# Autodesk Inventor assembly: mecanismo
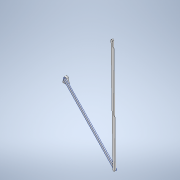
[picture p0: Inventor's stored thumbnail of the model, 180x180]
Saved by Autodesk Inventor 2021 (Build 250183000, 183)
## iProperties
Created: 2021-07-19
Part Number: mecanismo
Document SubType Name: Assembly
Designer: Leonardo Fabio Mercado Benítez
Author: Leonardo Fabio Mercado Benítez
## Documents named in this file (4)
- C:\Users\leo7s\Documents\Universidad\02 Servomecanismos\07 Proyecto Final\proyecto_final_Servomecanismos\02 CADs\mecanismo.iam
- C:\Users\leo7s\Documents\Universidad\02 Servomecanismos\07 Proyecto Final\proyecto_final_Servomecanismos\02 CADs\base.ipt
- C:\Users\leo7s\Documents\Universidad\02 Servomecanismos\07 Proyecto Final\proyecto_final_Servomecanismos\02 CADs\eslabon_1.ipt
- C:\Users\leo7s\Documents\Universidad\02 Servomecanismos\07 Proyecto Final\proyecto_final_Servomecanismos\02 CADs\eslasbon_2.ipt
## Components (3 placed, 3 different names)
1. base:1 — Coincidencia:1, Coincidencia:2, Coincidencia:3
2. eslabon_1:1 — Coincidencia:2, Coincidencia:3, Coincidencia:4, Coincidencia:5
3. eslasbon_2:1 — Coincidencia:4, Coincidencia:5
## Relationships (5: Mate 5)
- Coincidencia:1 [Mate]: base:1
- Coincidencia:2 [Mate]: base:1 ↔ eslabon_1:1
- Coincidencia:3 [Mate]: base:1 ↔ eslabon_1:1
- Coincidencia:4 [Mate]: eslabon_1:1 ↔ eslasbon_2:1
- Coincidencia:5 [Mate]: eslabon_1:1 ↔ eslasbon_2:1
